# Autodesk Inventor assembly: prostkatna waska niska kwadraty v2
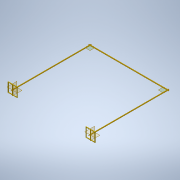
[picture p0: Inventor's stored thumbnail of the model, 180x180]
Saved by Autodesk Inventor 2021 (Build 250183000, 183)
## iProperties
Created: 2024-04-18
Part Number: prostkatna waska niska kwadraty v2
Document SubType Name: Assembly
Designer: Michal
Author: Michal
## Documents named in this file (5)
- C:\Users\Michal\Documents\GitHub\PNW_PhotoBoothFrame_3D\prostkatna waska niska kwadraty v2.iam
- C:\Users\Michal\Documents\GitHub\PNW_PhotoBoothFrame_3D\Stopa v1.iam
- C:\Users\Michal\Documents\GitHub\PNW_PhotoBoothFrame_3D\Lacznik prosty sruby.iam
- C:\Users\Michal\Documents\GitHub\PNW_PhotoBoothFrame_3D\Przedluzka L1500.ipt
- C:\Users\Michal\Documents\GitHub\PNW_PhotoBoothFrame_3D\Naroznik v2.iam
## Components (13 placed, 4 different names)
1. Stopa v1:1 [sub-assembly] — Flush:1, Flush:2, Mate:40, Flush:8, Flush:9
2. Stopa v1:2 [sub-assembly] — Flush:1, Flush:2, Mate:41, Flush:10, Flush:11
3. Lacznik prosty sruby:1 [sub-assembly] — Flush:12, Mate:42, Mate:43, Mate:49, Flush:13
4. Przedluzka L1500:1 — Mate:40, Flush:8, Flush:9, Flush:12, Mate:42, Mate:43, Mate:50
5. Przedluzka L1500:2 — Mate:41, Flush:10, Flush:11, Mate:44, Mate:45, Mate:46
6. Lacznik prosty sruby:2 [sub-assembly] — Mate:44, Mate:45, Mate:46, Mate:63, Mate:64, Mate:65
7. Naroznik v2:1 [sub-assembly] — Mate:47, Mate:48, Mate:51, Flush:61, Mate:61, Mate:62
8. Przedluzka L1500:3 — Mate:47, Mate:48, Mate:49, Mate:50, Flush:13, Mate:51
9. Lacznik prosty sruby:3 [sub-assembly]
10. Przedluzka L1500:4 — Flush:61, Mate:61, Mate:62
11. Naroznik v2:2 [sub-assembly] — Mate:59, Mate:66
12. Przedluzka L1500:5 — Mate:59
13. Przedluzka L1500:6 — Mate:63, Mate:64, Mate:65, Mate:66
## Relationships (36: Mate 25, Flush 11)
- Flush:1: Stopa v1:1 ↔ Stopa v1:2
- Flush:2: Stopa v1:1 ↔ Stopa v1:2
- Mate:40: Stopa v1:1 ↔ Przedluzka L1500:1
- Flush:8: Stopa v1:1 ↔ Przedluzka L1500:1
- Flush:9: Stopa v1:1 ↔ Przedluzka L1500:1
- Mate:41: Stopa v1:2 ↔ Przedluzka L1500:2
- Flush:10: Stopa v1:2 ↔ Przedluzka L1500:2
- Flush:11: Stopa v1:2 ↔ Przedluzka L1500:2
- Flush:12: Lacznik prosty sruby:1 ↔ Przedluzka L1500:1
- Mate:42: Lacznik prosty sruby:1 ↔ Przedluzka L1500:1
- Mate:43: Lacznik prosty sruby:1 ↔ Przedluzka L1500:1
- Mate:44: Przedluzka L1500:2 ↔ Lacznik prosty sruby:2
- Mate:45: Przedluzka L1500:2 ↔ Lacznik prosty sruby:2
- Mate:46: Przedluzka L1500:2 ↔ Lacznik prosty sruby:2
- Mate:47: Naroznik v2:1 ↔ Przedluzka L1500:3
- Mate:48: Naroznik v2:1 ↔ Przedluzka L1500:3
- Mate:49: Lacznik prosty sruby:1 ↔ Przedluzka L1500:3
- Mate:50: Przedluzka L1500:1 ↔ Przedluzka L1500:3
- Flush:13: Lacznik prosty sruby:1 ↔ Przedluzka L1500:3
- Mate:51: Naroznik v2:1 ↔ Przedluzka L1500:3
- [Flush]: Lacznik prosty sruby:3 ↔ Przedluzka L1500:4
- [Mate]: Lacznik prosty sruby:3 ↔ Przedluzka L1500:4
- [Mate]: Lacznik prosty sruby:3 ↔ Przedluzka L1500:4
- [Mate]: Naroznik v2:2 ↔ Przedluzka L1500:5
- [Mate]: Lacznik prosty sruby:3 ↔ Przedluzka L1500:5
- [Mate]: Przedluzka L1500:4 ↔ Przedluzka L1500:5
- [Flush]: Lacznik prosty sruby:3 ↔ Przedluzka L1500:5
- [Mate]: Naroznik v2:2 ↔ Przedluzka L1500:5
- Mate:59: Naroznik v2:2 ↔ Przedluzka L1500:5
- Flush:61: Naroznik v2:1 ↔ Przedluzka L1500:4
- Mate:61: Naroznik v2:1 ↔ Przedluzka L1500:4
- Mate:62: Naroznik v2:1 ↔ Przedluzka L1500:4
- Mate:63: Lacznik prosty sruby:2 ↔ Przedluzka L1500:6
- Mate:64: Lacznik prosty sruby:2 ↔ Przedluzka L1500:6
- Mate:65: Lacznik prosty sruby:2 ↔ Przedluzka L1500:6
- Mate:66: Naroznik v2:2 ↔ Przedluzka L1500:6
## Named parameters: d69_d56 = 0 mm, d70_d57 = 0 mm, d71_d63 = 0 mm, d73_d65 = 0 mm, d74_d66 = 0 mm, d75_d67 = 0 mm, d76_d68 = 0 mm, d77_d55 = 0 mm
